# Autodesk Inventor assembly: left_arm
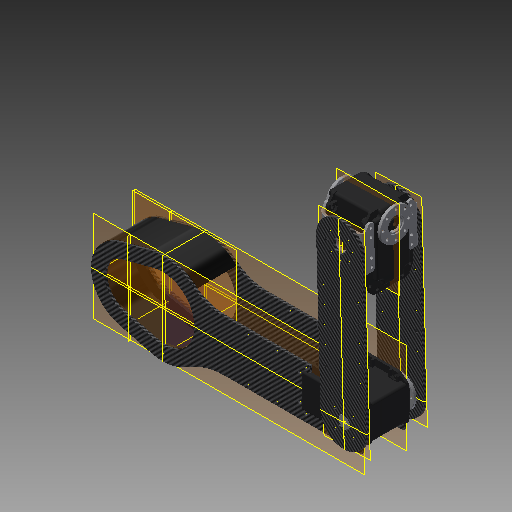
[picture p0: Inventor's stored thumbnail of the model, 512x512]
Saved by Autodesk Inventor 2018 (Build 220112000, 112)
## iProperties
Created: 2018-11-27
Part Number: left_arm
Document SubType Name: Assembly
Designer: bitbots
Author: bitbots
## Documents named in this file (6)
- C:\Users\jaspe\gitss\bitbots_hardware\wolfgang\assembly\arms\left_arm.iam
- C:\Users\jaspe\gitss\bitbots_hardware\wolfgang\assembly\arms\forearm.ipt
- C:\Users\jaspe\gitss\bitbots_hardware\wolfgang\assembly\motors\MX64\Mx64_with_bearing.iam
- C:\Users\jaspe\gitss\bitbots_hardware\wolfgang\assembly\arms\hand.ipt
- C:\Users\jaspe\gitss\bitbots_hardware\wolfgang\assembly\arms\upperarm.ipt
- C:\Users\jaspe\gitss\bitbots_hardware\wolfgang\assembly\arms\connector_shoulder.ipt
## Components (9 placed, 5 different names)
1. forearm:1 — Mate:1, Mate:2, Mate:3, Mate:10
2. forearm:2 — Mate:4, Mate:5, Mate:6, Mate:7, Mate:8, Mate:9
3. Mx64_with_bearing:1 [sub-assembly] — Mate:1, Mate:2, Mate:3, Mate:4, Mate:5, Mate:6, Mate:11, Mate:12, Mate:13, Mate:14, Mate:15
4. hand:1 — Mate:7, Mate:8, Mate:9, Mate:10
5. upperarm:1 — Mate:14, Mate:15, Mate:25
6. upperarm:2 — Mate:11, Mate:12, Mate:13, Mate:22, Mate:23, Mate:24
7. Mx64_with_bearing:2 [sub-assembly] — Mate:16, Mate:17, Mate:18, Mate:19, Mate:20, Mate:21, Flush:1
8. connector_shoulder:1 — Mate:19, Mate:20, Mate:21, Mate:22, Mate:23, Mate:24
9. connector_shoulder:2 — Mate:16, Mate:17, Mate:18, Mate:25
## Relationships (26: Mate 25, Flush 1)
- Mate:1: forearm:1 ↔ Mx64_with_bearing:1
- Mate:2: forearm:1 ↔ Mx64_with_bearing:1
- Mate:3: forearm:1 ↔ Mx64_with_bearing:1
- Mate:4: forearm:2 ↔ Mx64_with_bearing:1
- Mate:5: forearm:2 ↔ Mx64_with_bearing:1
- Mate:6: forearm:2 ↔ Mx64_with_bearing:1
- Mate:7: forearm:2 ↔ hand:1
- Mate:8: forearm:2 ↔ hand:1
- Mate:9: forearm:2 ↔ hand:1
- Mate:10: forearm:1 ↔ hand:1
- Mate:11: Mx64_with_bearing:1 ↔ upperarm:2
- Mate:12: Mx64_with_bearing:1 ↔ upperarm:2
- Mate:13: Mx64_with_bearing:1 ↔ upperarm:2
- Mate:14: Mx64_with_bearing:1 ↔ upperarm:1
- Mate:15: Mx64_with_bearing:1 ↔ upperarm:1
- Mate:16: Mx64_with_bearing:2 ↔ connector_shoulder:2
- Mate:17: Mx64_with_bearing:2 ↔ connector_shoulder:2
- Mate:18: Mx64_with_bearing:2 ↔ connector_shoulder:2
- Mate:19: Mx64_with_bearing:2 ↔ connector_shoulder:1
- Mate:20: Mx64_with_bearing:2 ↔ connector_shoulder:1
- Mate:21: Mx64_with_bearing:2 ↔ connector_shoulder:1
- Mate:22: upperarm:2 ↔ connector_shoulder:1
- Mate:23: upperarm:2 ↔ connector_shoulder:1
- Mate:24: upperarm:2 ↔ connector_shoulder:1
- Mate:25: upperarm:1 ↔ connector_shoulder:2
- Flush:1 (-14.5 mm): Mx64_with_bearing:2
